# Autodesk Inventor assembly: haptic_ass_1
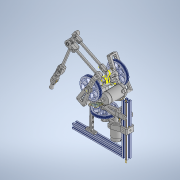
[picture p0: Inventor's stored thumbnail of the model, 180x180]
Saved by Autodesk Inventor 2020 (Build 240168000, 168)
## iProperties
Created: 2019-10-15
Part Number: haptic_ass_1
Document SubType Name: Assembly
Designer: psrob
Author: psrob
## Documents named in this file (24)
- E:\projects-2\haptic device gen3\hardware\haptic_ass_1.iam
- E:\projects-2\haptic device gen3\hardware\upper_arm_1.iam
- E:\projects-2\haptic device gen3\hardware\belt_reducer_2.iam
- E:\projects-2\haptic device gen3\hardware\armtip_1.ipt
- E:\projects-2\haptic device gen3\hardware\armtip_2.ipt
- E:\projects-2\haptic device gen3\hardware\carbon_fiber_1.ipt
- E:\projects-2\haptic device gen3\hardware\armtip_3.ipt
- E:\projects-2\haptic device gen3\hardware\bearing_6_13_5.ipt
- E:\projects-2\haptic device gen3\hardware\sub_arm_1.ipt
- E:\projects-2\haptic device gen3\hardware\sub_arm_2.ipt
- E:\projects-2\haptic device gen3\hardware\arm_linkage_1.ipt
- E:\projects-2\haptic device gen3\hardware\bearing_3_10_5.ipt
- E:\projects-2\haptic device gen3\hardware\arm_linkage_2.ipt
- E:\projects-2\haptic device gen3\hardware\arm_linkage_3.ipt
- E:\projects-2\haptic device gen3\hardware\2020_fixer_1.ipt
- E:\projects-2\haptic device gen3\hardware\2020.ipt
- E:\projects-2\haptic device gen3\hardware\2020_fixer2.ipt
- E:\projects-2\haptic device gen3\hardware\2200_support_3.ipt
- E:\projects-2\haptic device gen3\hardware\end_tip_1.ipt
- E:\projects-2\haptic device gen3\hardware\end_tip_2.ipt
- E:\projects-2\haptic device gen3\hardware\4_20.ipt
- E:\projects-2\haptic device gen3\hardware\bearing_4_9_5.ipt
- E:\projects-2\haptic device gen3\hardware\arm_tip_3.ipt
- E:\projects-2\haptic device gen3\hardware\arm_tip_4.ipt
## Components (34 placed, 23 different names)
1. upper_arm_1:1 [sub-assembly] — Insert:1, Insert:2, Insert:13
2. belt_reducer_2:1 [sub-assembly] — Insert:1, Insert:2, Insert:26, Insert:27, Flush:10, Flush:11
3. armtip_1:1 — Mate:1, Mate:2, Mate:3, Insert:4, Insert:5
4. armtip_2:1 — Insert:4, Insert:5
5. carbon_fiber_1:1 — Mate:1, Mate:2, Mate:3, Mate:4, Mate:5, Mate:6
6. armtip_3:1 — Insert:6, Insert:7, Insert:8
7. armtip_3:2 — Mate:4, Mate:5, Mate:6, Insert:6, Insert:7, Insert:9
8. bearing_6_13_5:1 — Insert:8, Insert:24
9. bearing_6_13_5:2 — Insert:9
10. sub_arm_1:1 — Mate:7, Mate:8, Mate:9, Flush:2, Insert:11, Insert:12, Insert:14, Insert:15, Insert:24, Insert:25
11. carbon_fiber_1:2 — Mate:7, Mate:8, Mate:9, Flush:12, Mate:20, Mate:21, Mate:22
12. sub_arm_2:1 — Flush:2, Insert:11, Insert:12, Angle:1
13. arm_linkage_1:1 — Insert:13, Insert:16, Insert:17, Angle:1
14. bearing_3_10_5:1 — Insert:14
15. bearing_3_10_5:2 — Insert:15
16. bearing_3_10_5:3 — Insert:16, Insert:19
17. bearing_3_10_5:4 — Insert:17
18. arm_linkage_2:1 — Mate:10, Mate:11, Mate:12, Insert:22, Insert:23, Insert:25
19. arm_linkage_2:2 — Insert:19, Mate:13, Mate:14, Flush:4, Insert:20, Insert:21
20. carbon_fiber_1:3 — Mate:10, Mate:11, Mate:12, Mate:13, Mate:14, Mate:15
21. arm_linkage_3:1 — Flush:4, Insert:20, Insert:21, Mate:15
22. arm_linkage_3:2 — Insert:22, Insert:23
23. 2020_fixer_1:1 — Insert:26, Insert:27, Mate:16, Mate:17, Flush:5
24. 2020:1 — Mate:16, Mate:17, Flush:5, Mate:19, Flush:6, Flush:7, Flush:8, Flush:9
25. 2020:2 — Mate:19, Flush:6, Flush:7
26. 2020_fixer2:1 — Flush:8, Flush:9, Flush:10
27. 2200_support_3:1 — Flush:11
28. end_tip_1:1 — Flush:12, Flush:13, Mate:20, Mate:21, Mate:22, Insert:28, Insert:29, Insert:30, Insert:31, Flush:14, Angle:2
29. end_tip_2:1 — Flush:13, Insert:28, Insert:29
30. 4_20:1 — Insert:30, Insert:32
31. bearing_4_9_5:1 — Insert:31, Insert:33
32. bearing_4_9_5:2 — Insert:32
33. arm_tip_3:1 — Flush:14, Insert:33, Angle:2, Flush:15
34. arm_tip_4:1 — Flush:15
## Relationships (66: Insert 30, Mate 21, Flush 13, Angle 2)
- Insert:1: upper_arm_1:1 ↔ belt_reducer_2:1
- Insert:2: upper_arm_1:1 ↔ belt_reducer_2:1
- Mate:1: armtip_1:1 ↔ carbon_fiber_1:1
- Mate:2: armtip_1:1 ↔ carbon_fiber_1:1
- Mate:3: armtip_1:1 ↔ carbon_fiber_1:1
- Insert:4: armtip_1:1 ↔ armtip_2:1
- Insert:5: armtip_1:1 ↔ armtip_2:1
- Mate:4: carbon_fiber_1:1 ↔ armtip_3:2
- Mate:5: carbon_fiber_1:1 ↔ armtip_3:2
- Mate:6: carbon_fiber_1:1 ↔ armtip_3:2
- Insert:6: armtip_3:1 ↔ armtip_3:2
- Insert:7: armtip_3:1 ↔ armtip_3:2
- Insert:8: armtip_3:1 ↔ bearing_6_13_5:1
- Insert:9: armtip_3:2 ↔ bearing_6_13_5:2
- Mate:7: sub_arm_1:1 ↔ carbon_fiber_1:2
- Mate:8: sub_arm_1:1 ↔ carbon_fiber_1:2
- Mate:9: sub_arm_1:1 ↔ carbon_fiber_1:2
- Flush:2: sub_arm_1:1 ↔ sub_arm_2:1
- Insert:11: sub_arm_1:1 ↔ sub_arm_2:1
- Insert:12: sub_arm_1:1 ↔ sub_arm_2:1
- Insert:13 (-5 mm): upper_arm_1:1 ↔ arm_linkage_1:1
- Insert:14: sub_arm_1:1 ↔ bearing_3_10_5:1
- Insert:15: sub_arm_1:1 ↔ bearing_3_10_5:2
- Insert:16: arm_linkage_1:1 ↔ bearing_3_10_5:3
- Insert:17: arm_linkage_1:1 ↔ bearing_3_10_5:4
- Angle:1 (0 deg): sub_arm_2:1 ↔ arm_linkage_1:1
- Insert:19: bearing_3_10_5:3 ↔ arm_linkage_2:2
- Mate:10: arm_linkage_2:1 ↔ carbon_fiber_1:3
- Mate:11: arm_linkage_2:1 ↔ carbon_fiber_1:3
- Mate:12: arm_linkage_2:1 ↔ carbon_fiber_1:3
- Mate:13: arm_linkage_2:2 ↔ carbon_fiber_1:3
- Mate:14: arm_linkage_2:2 ↔ carbon_fiber_1:3
- Flush:4: arm_linkage_2:2 ↔ arm_linkage_3:1
- Insert:20: arm_linkage_2:2 ↔ arm_linkage_3:1
- Insert:21: arm_linkage_2:2 ↔ arm_linkage_3:1
- Insert:22: arm_linkage_2:1 ↔ arm_linkage_3:2
- Insert:23: arm_linkage_2:1 ↔ arm_linkage_3:2
- Insert:24: bearing_6_13_5:1 ↔ sub_arm_1:1
- Mate:15: carbon_fiber_1:3 ↔ arm_linkage_3:1
- Insert:25: sub_arm_1:1 ↔ arm_linkage_2:1
- Insert:26: belt_reducer_2:1 ↔ 2020_fixer_1:1
- Insert:27: belt_reducer_2:1 ↔ 2020_fixer_1:1
- Mate:16: 2020_fixer_1:1 ↔ 2020:1
- Mate:17 (-60 mm): 2020_fixer_1:1 ↔ 2020:1
- Flush:5: 2020_fixer_1:1 ↔ 2020:1
- Mate:19: 2020:1 ↔ 2020:2
- Flush:6: 2020:1 ↔ 2020:2
- Flush:7: 2020:1 ↔ 2020:2
- Flush:8: 2020:1 ↔ 2020_fixer2:1
- Flush:9: 2020:1 ↔ 2020_fixer2:1
- Flush:10: belt_reducer_2:1 ↔ 2020_fixer2:1
- Flush:11: belt_reducer_2:1 ↔ 2200_support_3:1
- Flush:12: carbon_fiber_1:2 ↔ end_tip_1:1
- Flush:13: end_tip_1:1 ↔ end_tip_2:1
- Mate:20: carbon_fiber_1:2 ↔ end_tip_1:1
- Mate:21: carbon_fiber_1:2 ↔ end_tip_1:1
- Mate:22: carbon_fiber_1:2 ↔ end_tip_1:1
- Insert:28: end_tip_1:1 ↔ end_tip_2:1
- Insert:29: end_tip_1:1 ↔ end_tip_2:1
- Insert:30: end_tip_1:1 ↔ 4_20:1
- Insert:31: end_tip_1:1 ↔ bearing_4_9_5:1
- Insert:32: 4_20:1 ↔ bearing_4_9_5:2
- Flush:14: end_tip_1:1 ↔ arm_tip_3:1
- Insert:33: bearing_4_9_5:1 ↔ arm_tip_3:1
- Angle:2 (0 deg): end_tip_1:1 ↔ arm_tip_3:1
- Flush:15: arm_tip_3:1 ↔ arm_tip_4:1
